# Autodesk Inventor assembly: Assembly
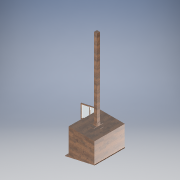
[picture p0: Inventor's stored thumbnail of the model, 180x180]
Saved by Autodesk Inventor 2017 (Build 210142000, 142)
## iProperties
Created: 2016-09-08
Part Number: Assembly
Document SubType Name: Assembly
Designer: s.ethan.wierenga
Author: s.ethan.wierenga
## Documents named in this file (5)
- E:\Github\home\ahri\.freepantry\.files\Assembly.iam
- E:\Github\home\ahri\.freepantry\.files\Post Bracket.ipt
- E:\Github\home\ahri\.freepantry\.files\Post Stick.ipt
- E:\Github\home\ahri\.freepantry\.files\Top.ipt
- E:\Github\home\ahri\.freepantry\.files\Full Door.iam
## Components (8 placed, 4 different names)
1. Post Bracket:1 — Flush:7, Mate:4, Flush:8, Flush:9
2. Post Stick:1 — Flush:1, Mate:1, Flush:2, Flush:3, Mate:2, Flush:4, Flush:5, Mate:3, Flush:6, Flush:7, Mate:4, Flush:8, Mate:5
3. Post Bracket:2 — Flush:5, Mate:3, Flush:6
4. Post Bracket:3 — Flush:1, Mate:1, Flush:2
5. Post Bracket:4 — Flush:3, Mate:2, Flush:4, Flush:10
6. Top:1 — Flush:9, Mate:5, Flush:10, Mate:6, Flush:11, Mate:7, Flush:12
7. Full Door:1 [sub-assembly] — Mate:6, Flush:11
8. Full Door:2 [sub-assembly] — Mate:7, Flush:12
## Relationships (19: Flush 12, Mate 7)
- Flush:1: Post Stick:1 ↔ Post Bracket:3
- Mate:1: Post Stick:1 ↔ Post Bracket:3
- Flush:2: Post Stick:1 ↔ Post Bracket:3
- Flush:3: Post Stick:1 ↔ Post Bracket:4
- Mate:2: Post Stick:1 ↔ Post Bracket:4
- Flush:4: Post Stick:1 ↔ Post Bracket:4
- Flush:5: Post Stick:1 ↔ Post Bracket:2
- Mate:3: Post Stick:1 ↔ Post Bracket:2
- Flush:6: Post Stick:1 ↔ Post Bracket:2
- Flush:7: Post Bracket:1 ↔ Post Stick:1
- Mate:4: Post Bracket:1 ↔ Post Stick:1
- Flush:8: Post Bracket:1 ↔ Post Stick:1
- Flush:9 (311.15 mm): Post Bracket:1 ↔ Top:1
- Mate:5: Post Stick:1 ↔ Top:1
- Flush:10 (234.95 mm): Post Bracket:4 ↔ Top:1
- Mate:6: Top:1 ↔ Full Door:1
- Flush:11: Top:1 ↔ Full Door:1
- Mate:7: Top:1 ↔ Full Door:2
- Flush:12: Top:1 ↔ Full Door:2
